# Autodesk Inventor assembly: assy-shooter_light
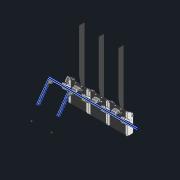
[picture p0: Inventor's stored thumbnail of the model, 180x180]
Saved by Autodesk Inventor 2022 (Build 260153000, 153)
## iProperties
Created: 2021-08-20
Part Number: assy-shooter_light
Document SubType Name: Assembly
Designer: yuta0
Mass: 3165.35 g
Surface Area: 11091.2 cm^2
Volume: 1829.85 cm^3
Density: 1.72984 g/cm^3
Author: yuta0
## Documents named in this file (18)
- C:\Users\yuta0\Documents\GitHub\catchrobo_hardware\assy-shooter\assy-shooter_light.iam
- C:\Users\yuta0\Documents\GitHub\catchrobo_hardware\assy-shooter\shooter_carbon_plate1.ipt
- C:\Users\yuta0\Documents\GitHub\catchrobo_hardware\assy-shooter\shooter_base4.ipt
- C:\Users\yuta0\Documents\GitHub\catchrobo_hardware\assy-shooter\MF126ZZ.ipt
- C:\Users\yuta0\Documents\GitHub\catchrobo_hardware\assy-shooter\s-assy-sorter_motor.iam
- C:\Users\yuta0\Documents\GitHub\catchrobo_hardware\assy-shooter\s-assy-shooter_motor2.iam
- C:\Users\yuta0\Documents\GitHub\catchrobo_hardware\assy-shooter\s-assy-sorter_plate.iam
- C:\Users\yuta0\Documents\GitHub\catchrobo_hardware\assy-shooter\s-assy-guide_plates.iam
- C:\Users\yuta0\Documents\GitHub\catchrobo_hardware\assy-shooter\CBSTSR3-10.ipt
- C:\Users\yuta0\Documents\GitHub\catchrobo_hardware\assy-shooter\LBNR3.ipt
- C:\Users\yuta0\Documents\GitHub\catchrobo_hardware\assy-shooter\CB3-15.ipt
- C:\Users\yuta0\Documents\GitHub\catchrobo_hardware\assy-shooter\shooter_base1.ipt
- C:\Users\yuta0\Documents\GitHub\catchrobo_hardware\assy-shooter\s-assy-frame-connector.iam
- C:\Users\yuta0\Documents\GitHub\catchrobo_hardware\assy-shooter\s-assy-bearing_stopper.iam
- C:\Users\yuta0\Documents\GitHub\catchrobo_hardware\assy-shooter\d_type_board.ipt
- C:\Users\yuta0\Documents\GitHub\catchrobo_hardware\assy-shooter\hexagonal_spacer_M3_5mm.ipt
- C:\Users\yuta0\Documents\GitHub\catchrobo_hardware\assy-shooter\CB3-5.ipt
- C:\Users\yuta0\Documents\GitHub\catchrobo_hardware\assy-shooter\s-assy-shooter_frame_light.iam
## Components (94 placed, 17 different names)
1. s-assy-shooter_motor2:1 [sub-assembly] — メイト:215, メイト:222, メイト:280, メイト:282, メイト:283
2. s-assy-guide_plates:1 [sub-assembly] — メイト:222, 角度:2, メイト:280, メイト:285, メイト:293
3. s-assy-bearing_stopper:7 [sub-assembly] — メイト:279
4. MF126ZZ:2 — メイト:56, メイト:281
5. MF126ZZ:9 — メイト:279
6. d_type_board:1 — メイト:299, メイト:300
7. s-assy-shooter_frame_light:1 [sub-assembly] — メイト:301, メイト:302, フラッシュ:10, メイト:304, メイト:305
8. s-assy-frame-connector:3 [sub-assembly] — メイト:271, メイト:292, メイト:301, メイト:302, メイト:303
9. s-assy-frame-connector:4 [sub-assembly] — メイト:296, メイト:297
10. s-assy-frame-connector:5 [sub-assembly]
11. s-assy-frame-connector:6 [sub-assembly] — メイト:304, メイト:305
12. shooter_carbon_plate1:1 — メイト:20, メイト:21, フラッシュ:6, メイト:209, メイト:210, メイト:212, メイト:223, メイト:224, メイト:250, メイト:284, メイト:286, メイト:287
13. shooter_base4:1 — メイト:20, メイト:21, フラッシュ:6, メイト:53, メイト:54, メイト:56, メイト:215, メイト:226, メイト:271, メイト:281, メイト:282, メイト:283, フラッシュ:10
14. shooter_base1:1 — メイト:248, メイト:249, メイト:250, メイト:252, 角度:3, メイト:256, メイト:257, メイト:258, メイト:260, メイト:261, メイト:284
15. s-assy-sorter_plate:1 [sub-assembly] — メイト:217, メイト:218, 角度:1
16. s-assy-sorter_motor:1 [sub-assembly] — メイト:209, メイト:210, メイト:212, メイト:217, メイト:218, 角度:1
17. s-assy-bearing_stopper:2 [sub-assembly] — メイト:277, メイト:293
18. MF126ZZ:4 — メイト:252, メイト:277, メイト:285
19. s-assy-bearing_stopper:1 [sub-assembly] — メイト:275
20. MF126ZZ:1 — メイト:53, メイト:54, メイト:275
21. shooter_carbon_plate1:2
22. shooter_base4:2 — メイト:288, メイト:289, メイト:290, メイト:291
23. shooter_base1:2
24. s-assy-sorter_plate:2 [sub-assembly]
25. s-assy-sorter_motor:2 [sub-assembly]
26. s-assy-bearing_stopper:8 [sub-assembly]
27. MF126ZZ:10
28. s-assy-bearing_stopper:10 [sub-assembly]
29. MF126ZZ:12
30. shooter_carbon_plate1:3
31. shooter_base4:3
32. shooter_base1:3
33. s-assy-sorter_plate:3 [sub-assembly]
34. s-assy-sorter_motor:3 [sub-assembly]
35. s-assy-bearing_stopper:9 [sub-assembly]
36. MF126ZZ:11
37. s-assy-bearing_stopper:11 [sub-assembly]
38. MF126ZZ:13
39. LBNR3:18 — メイト:247, 角度:3, 角度:4, フラッシュ:9
40. LBNR3:17 — メイト:245, 角度:4, 角度:5, フラッシュ:8, フラッシュ:9
41. LBNR3:16 — メイト:243, 角度:6, フラッシュ:7, フラッシュ:8, メイト:256
42. LBNR3:15 — メイト:241, 角度:5, 角度:6, フラッシュ:7
43. CB3-15:4 — メイト:241, メイト:257, メイト:289
44. CB3-15:3 — メイト:243, メイト:261, メイト:288
45. CB3-15:2 — メイト:247, メイト:260, メイト:291
46. CB3-15:1 — メイト:245, メイト:258, メイト:290
47. LBNR3:27
48. LBNR3:28
49. LBNR3:29
50. LBNR3:30
51. CB3-15:5
52. CB3-15:6
53. CB3-15:7
54. CB3-15:8
55. hexagonal_spacer_M3_5mm:1 — メイト:296, メイト:297
56. CB3-5:1 — メイト:299, メイト:300
57. hexagonal_spacer_M3_5mm:2
58. CB3-5:2
59. CBSTSR3-10:1 — メイト:223, メイト:224, メイト:225
60. LBNR3:1 — メイト:225, メイト:226
61. CBSTSR3-10:2
62. LBNR3:2
63. CBSTSR3-10:3 — メイト:248
64. LBNR3:3
65. CBSTSR3-10:4 — メイト:249
66. LBNR3:4
67. CBSTSR3-10:5 — メイト:286, メイト:287, メイト:292
68. CBSTSR3-10:6 — メイト:303
69. CBSTSR3-10:7
70. CBSTSR3-10:8
71. CBSTSR3-10:9
72. LBNR3:19
73. CBSTSR3-10:10
74. LBNR3:20
75. CBSTSR3-10:11
76. LBNR3:21
77. CBSTSR3-10:12
78. LBNR3:22
79. CBSTSR3-10:13
80. CBSTSR3-10:14
81. CBSTSR3-10:15
82. CBSTSR3-10:16
83. CBSTSR3-10:17
84. LBNR3:23
85. CBSTSR3-10:18
86. LBNR3:24
87. CBSTSR3-10:19
88. LBNR3:25
89. CBSTSR3-10:20
90. LBNR3:26
91. CBSTSR3-10:21
92. CBSTSR3-10:22
93. CBSTSR3-10:23
94. CBSTSR3-10:24
## Component patterns: (4 elements, first: s-assy-frame-connector:3), (3 elements, first: shooter_carbon_plate1:1 + shooter_base4:1 + shooter_base1:1 + s-assy-sorter_plate:1 + s-assy-sorter_motor:1 + s-assy-bearing_stopper:2 + MF126ZZ:4 + s-assy-bearing_stopper:1 + MF126ZZ:1), (2 elements, first: LBNR3:18 + LBNR3:17 + LBNR3:16 + LBNR3:15 + CB3-15:4 + CB3-15:3 + CB3-15:2 + CB3-15:1), (2 elements, first: hexagonal_spacer_M3_5mm:1 + CB3-5:1), (4 elements, first: CBSTSR3-10:1 + LBNR3:1), (4 elements, first: CBSTSR3-10:5), コンポーネント パターン 4:2 (4 elements), コンポーネント パターン 12:2 (4 elements), コンポーネント パターン 4:3 (4 elements), コンポーネント パターン 12:3 (4 elements)
## Relationships (67: Mate 56, Angle 6, Flush 5)
- 角度:1 [Angle] (0 deg): s-assy-sorter_plate:1 ↔ s-assy-sorter_motor:1
- 角度:2 [Angle] (0 deg): s-assy-guide_plates:1
- メイト:20 [Mate]: shooter_carbon_plate1:1 ↔ shooter_base4:1
- メイト:21 [Mate]: shooter_carbon_plate1:1 ↔ shooter_base4:1
- フラッシュ:6 [Flush]: shooter_carbon_plate1:1 ↔ shooter_base4:1
- メイト:53 [Mate]: shooter_base4:1 ↔ MF126ZZ:1
- メイト:54 [Mate]: shooter_base4:1 ↔ MF126ZZ:1
- メイト:56 [Mate]: MF126ZZ:2 ↔ shooter_base4:1
- メイト:209 [Mate]: shooter_carbon_plate1:1 ↔ s-assy-sorter_motor:1
- メイト:210 [Mate]: shooter_carbon_plate1:1 ↔ s-assy-sorter_motor:1
- メイト:212 [Mate]: shooter_carbon_plate1:1 ↔ s-assy-sorter_motor:1
- メイト:215 [Mate]: s-assy-shooter_motor2:1 ↔ shooter_base4:1
- メイト:217 [Mate]: s-assy-sorter_plate:1 ↔ s-assy-sorter_motor:1
- メイト:218 [Mate]: s-assy-sorter_plate:1 ↔ s-assy-sorter_motor:1
- メイト:222 [Mate]: s-assy-shooter_motor2:1 ↔ s-assy-guide_plates:1
- メイト:223 [Mate]: shooter_carbon_plate1:1 ↔ CBSTSR3-10:1
- メイト:224 [Mate]: shooter_carbon_plate1:1 ↔ CBSTSR3-10:1
- メイト:225 [Mate]: CBSTSR3-10:1 ↔ LBNR3:1
- メイト:226 [Mate]: shooter_base4:1 ↔ LBNR3:1
- メイト:241 [Mate]: LBNR3:15 ↔ CB3-15:4
- メイト:243 [Mate]: LBNR3:16 ↔ CB3-15:3
- メイト:245 [Mate]: LBNR3:17 ↔ CB3-15:1
- メイト:247 [Mate]: LBNR3:18 ↔ CB3-15:2
- メイト:248 [Mate]: shooter_base1:1 ↔ CBSTSR3-10:3
- メイト:249 [Mate]: shooter_base1:1 ↔ CBSTSR3-10:4
- メイト:250 [Mate]: shooter_carbon_plate1:1 ↔ shooter_base1:1
- メイト:252 [Mate]: shooter_base1:1 ↔ MF126ZZ:4
- 角度:3 [Angle] (0 deg): shooter_base1:1 ↔ LBNR3:18
- 角度:4 [Angle] (0 deg): LBNR3:18 ↔ LBNR3:17
- 角度:5 [Angle] (0 deg): LBNR3:17 ↔ LBNR3:15
- 角度:6 [Angle] (0 deg): LBNR3:16 ↔ LBNR3:15
- フラッシュ:7 [Flush]: LBNR3:16 ↔ LBNR3:15
- フラッシュ:8 [Flush]: LBNR3:17 ↔ LBNR3:16
- フラッシュ:9 [Flush]: LBNR3:18 ↔ LBNR3:17
- メイト:256 [Mate]: shooter_base1:1 ↔ LBNR3:16
- メイト:257 [Mate]: shooter_base1:1 ↔ CB3-15:4
- メイト:258 [Mate]: shooter_base1:1 ↔ CB3-15:1
- メイト:260 [Mate]: shooter_base1:1 ↔ CB3-15:2
- メイト:261 [Mate]: shooter_base1:1 ↔ CB3-15:3
- メイト:271 [Mate]: s-assy-frame-connector:3 ↔ shooter_base4:1
- メイト:275 [Mate]: s-assy-bearing_stopper:1 ↔ MF126ZZ:1
- メイト:277 [Mate]: s-assy-bearing_stopper:2 ↔ MF126ZZ:4
- メイト:279 [Mate]: s-assy-bearing_stopper:7 ↔ MF126ZZ:9
- メイト:280 [Mate]: s-assy-shooter_motor2:1 ↔ s-assy-guide_plates:1
- メイト:281 [Mate]: MF126ZZ:2 ↔ shooter_base4:1
- メイト:282 [Mate]: s-assy-shooter_motor2:1 ↔ shooter_base4:1
- メイト:283 [Mate]: s-assy-shooter_motor2:1 ↔ shooter_base4:1
- メイト:284 [Mate]: shooter_carbon_plate1:1 ↔ shooter_base1:1
- メイト:285 [Mate]: s-assy-guide_plates:1 ↔ MF126ZZ:4
- メイト:286 [Mate]: shooter_carbon_plate1:1 ↔ CBSTSR3-10:5
- メイト:287 [Mate]: shooter_carbon_plate1:1 ↔ CBSTSR3-10:5
- メイト:288 [Mate]: shooter_base4:2 ↔ CB3-15:3
- メイト:289 [Mate]: shooter_base4:2 ↔ CB3-15:4
- メイト:290 [Mate]: shooter_base4:2 ↔ CB3-15:1
- メイト:291 [Mate]: shooter_base4:2 ↔ CB3-15:2
- メイト:292 [Mate]: s-assy-frame-connector:3 ↔ CBSTSR3-10:5
- メイト:293 [Mate]: s-assy-guide_plates:1 ↔ s-assy-bearing_stopper:2
- メイト:296 [Mate]: s-assy-frame-connector:4 ↔ hexagonal_spacer_M3_5mm:1
- メイト:297 [Mate]: s-assy-frame-connector:4 ↔ hexagonal_spacer_M3_5mm:1
- メイト:299 [Mate]: d_type_board:1 ↔ CB3-5:1
- メイト:300 [Mate]: d_type_board:1 ↔ CB3-5:1
- メイト:301 [Mate]: s-assy-shooter_frame_light:1 ↔ s-assy-frame-connector:3
- メイト:302 [Mate]: s-assy-shooter_frame_light:1 ↔ s-assy-frame-connector:3
- メイト:303 [Mate]: s-assy-frame-connector:3 ↔ CBSTSR3-10:6
- フラッシュ:10 [Flush] (150 mm): s-assy-shooter_frame_light:1 ↔ shooter_base4:1
- メイト:304 [Mate]: s-assy-shooter_frame_light:1 ↔ s-assy-frame-connector:6
- メイト:305 [Mate]: s-assy-shooter_frame_light:1 ↔ s-assy-frame-connector:6
